# Autodesk Inventor assembly: Nema17
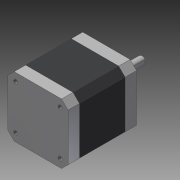
[picture p0: Inventor's stored thumbnail of the model, 180x180]
Saved by Autodesk Inventor 2014 SP1 (Build 180222100, 222)
## iProperties
Created: 2017-07-08
Part Number: Nema17
Document SubType Name: Assembly
Designer: Stepan
Author: Stepan
## Documents named in this file (5)
- D:\3DPrinter\Nema17\Nema17.iam
- D:\3DPrinter\Nema17\Axis.ipt
- D:\3DPrinter\Nema17\Body.ipt
- D:\3DPrinter\Nema17\Bottom.ipt
- D:\3DPrinter\Nema17\Top.ipt
## Components (4 placed, 4 different names)
1. Axis:1 — Совмещение:3
2. Body:1 — Совмещение:1, Совмещение:2, Заподлицо:1, Заподлицо:2, Заподлицо:3, Заподлицо:4
3. Bottom:1 — Совмещение:1, Заподлицо:3, Заподлицо:4
4. Top:1 — Совмещение:2, Заподлицо:1, Заподлицо:2, Совмещение:3
## Relationships (7: Flush 4, Mate 3)
- Совмещение:1 [Mate]: Body:1 ↔ Bottom:1
- Совмещение:2 [Mate]: Body:1 ↔ Top:1
- Заподлицо:1 [Flush]: Body:1 ↔ Top:1
- Заподлицо:2 [Flush]: Body:1 ↔ Top:1
- Заподлицо:3 [Flush]: Body:1 ↔ Bottom:1
- Заподлицо:4 [Flush]: Body:1 ↔ Bottom:1
- Совмещение:3 [Mate]: Axis:1 ↔ Top:1
